# Autodesk Inventor assembly: suspensionUnitMirrored
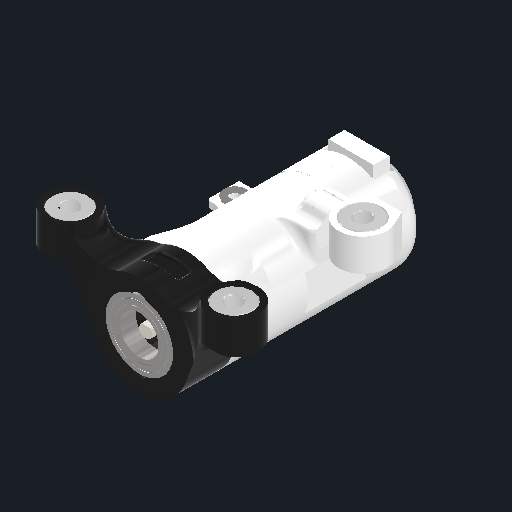
[picture p0: Inventor's stored thumbnail of the model, 512x512]
Saved by Autodesk Inventor 2025 (Build 290162000, 162)
## iProperties
Created: 2023-07-03
Part Number: suspensionUnitMirrored
Document SubType Name: Assembly
Designer: khrip
Mass: 81.1486 g
Surface Area: 305.3 cm^2
Volume: 59.2334 cm^3
Density: 1.36998 g/cm^3
Author: khrip
## Documents named in this file (13)
- H:\Potamon\OutdatedVersions\suspensionUnit\suspensionUnitMirrored.iam
- H:\Potamon\OutdatedVersions\suspensionUnit\servo.ipt
- H:\Potamon\OutdatedVersions\suspensionUnit\servoCushion.ipt
- H:\Potamon\OutdatedVersions\suspensionUnit\servoCushionSleeveMirrored.ipt
- C:\Users\khrip\OneDrive\Документы\Inventor\Content Center Files\R2023\ru-RU\GOST 17475-80 (2)\Винт 2.M3-6gx12 ГОСТ 17475-80.ipt
- H:\Potamon\OutdatedVersions\suspensionUnit\sleeve.ipt
- C:\Users\khrip\OneDrive\Документы\Inventor\Content Center Files\R2023\ru-RU\BS EN ISO 7045 H\EN ISO 7045 - M3 x 10 - 4.8 - H(1).ipt
- C:\Users\khrip\Documents\Inventor\Content Center Files\R2025\ru-RU\GOST 11371-78  A\Шайба 3 ГОСТ 11371-78.ipt
- C:\Users\khrip\OneDrive\Документы\Inventor\Content Center Files\R2023\ru-RU\DIN 934\DIN 934 - M3 x 0,5.ipt
- H:\Potamon\OutdatedVersions\suspensionUnit\bearing.ipt
- C:\Users\khrip\OneDrive\Документы\Inventor\Content Center Files\R2023\ru-RU\DIN 913\DIN 913 - M3 x 4.ipt
- H:\Potamon\OutdatedVersions\suspensionUnit\EncCoverHalf.ipt
- H:\Potamon\OutdatedVersions\suspensionUnit\EncCoverHalfMirrored.ipt
## Components (15 placed, 12 different names)
1. servo:1 — Совмещение:3, Совмещение:5, Совмещение:6, Совмещение:7, Совмещение:27, Совмещение:28, Угол:1, Совмещение:30
2. servoCushion:1 — Совмещение:1, Совмещение:2, Совмещение:4, Совмещение:5, Совмещение:6, Совмещение:7, Совмещение:8, Совмещение:9, Совмещение:12, Совмещение:13, Совмещение:14, Совмещение:15, Совмещение:22, Совмещение:23
3. servoCushionSleeveMirroredMirrored:1 — Совмещение:1, Совмещение:2, Совмещение:3, Совмещение:4, Совмещение:10, Совмещение:11, Совмещение:16, Совмещение:17, Совмещение:19, Совмещение:29, Совмещение:32
4. Винт 2 ГОСТ 17475-80 M3 x 12:1 — Совмещение:8
5. Винт 2 ГОСТ 17475-80 M3 x 12:2 — Совмещение:9
6. sleeve:1 — Совмещение:12, Совмещение:13
7. sleeve:2 — Совмещение:14, Совмещение:15
8. sleeve:3 — Совмещение:10, Совмещение:11
9. BS EN ISO 7045 H - метрическая M3 x 10 - 4.8 - H:1 — Совмещение:16, Совмещение:17, Совмещение:18, Совмещение:20
10. Шайба  ГОСТ 11371-78 3,2:1 — Совмещение:18, Совмещение:19, Совмещение:21
11. DIN 934 - заменено на DIN EN 24032/28673/28674 M3:1 — Совмещение:20, Совмещение:21
12. bearing:1 — Совмещение:22, Совмещение:23
13. DIN 913 M3 x 4:1 — Совмещение:27
14. EncCoverHalf:1 — Совмещение:28, Угол:1, Совмещение:29, Совмещение:31
15. EncCoverHalfMirrored:1 — Совмещение:30, Совмещение:31, Совмещение:32
## Relationships (30: Mate 29, Angle 1)
- Совмещение:1 [Mate]: servoCushion:1 ↔ servoCushionSleeveMirroredMirrored:1
- Совмещение:2 [Mate]: servoCushion:1 ↔ servoCushionSleeveMirroredMirrored:1
- Совмещение:3 [Mate]: servo:1 ↔ servoCushionSleeveMirroredMirrored:1
- Совмещение:4 [Mate]: servoCushion:1 ↔ servoCushionSleeveMirroredMirrored:1
- Совмещение:5 [Mate]: servo:1 ↔ servoCushion:1
- Совмещение:6 [Mate]: servo:1 ↔ servoCushion:1
- Совмещение:7 [Mate]: servo:1 ↔ servoCushion:1
- Совмещение:8 [Mate]: servoCushion:1 ↔ Винт 2 ГОСТ 17475-80 M3 x 12:1
- Совмещение:9 [Mate]: servoCushion:1 ↔ Винт 2 ГОСТ 17475-80 M3 x 12:2
- Совмещение:10 [Mate]: servoCushionSleeveMirroredMirrored:1 ↔ sleeve:3
- Совмещение:11 [Mate]: servoCushionSleeveMirroredMirrored:1 ↔ sleeve:3
- Совмещение:12 [Mate]: servoCushion:1 ↔ sleeve:1
- Совмещение:13 [Mate]: servoCushion:1 ↔ sleeve:1
- Совмещение:14 [Mate]: servoCushion:1 ↔ sleeve:2
- Совмещение:15 [Mate]: servoCushion:1 ↔ sleeve:2
- Совмещение:16 [Mate]: servoCushionSleeveMirroredMirrored:1 ↔ BS EN ISO 7045 H - метрическая M3 x 10 - 4.8 - H:1
- Совмещение:17 [Mate]: servoCushionSleeveMirroredMirrored:1 ↔ BS EN ISO 7045 H - метрическая M3 x 10 - 4.8 - H:1
- Совмещение:18 [Mate]: BS EN ISO 7045 H - метрическая M3 x 10 - 4.8 - H:1 ↔ Шайба  ГОСТ 11371-78 3,2:1
- Совмещение:19 [Mate]: servoCushionSleeveMirroredMirrored:1 ↔ Шайба  ГОСТ 11371-78 3,2:1
- Совмещение:20 [Mate]: BS EN ISO 7045 H - метрическая M3 x 10 - 4.8 - H:1 ↔ DIN 934 - заменено на DIN EN 24032/28673/28674 M3:1
- Совмещение:21 [Mate]: Шайба  ГОСТ 11371-78 3,2:1 ↔ DIN 934 - заменено на DIN EN 24032/28673/28674 M3:1
- Совмещение:22 [Mate]: servoCushion:1 ↔ bearing:1
- Совмещение:23 [Mate]: servoCushion:1 ↔ bearing:1
- Совмещение:27 [Mate]: servo:1 ↔ DIN 913 M3 x 4:1
- Совмещение:28 [Mate]: servo:1 ↔ EncCoverHalf:1
- Угол:1 [Angle] (180 deg): servo:1 ↔ EncCoverHalf:1
- Совмещение:29 [Mate]: servoCushionSleeveMirroredMirrored:1 ↔ EncCoverHalf:1
- Совмещение:30 [Mate]: servo:1 ↔ EncCoverHalfMirrored:1
- Совмещение:31 [Mate]: EncCoverHalf:1 ↔ EncCoverHalfMirrored:1
- Совмещение:32 [Mate]: servoCushionSleeveMirroredMirrored:1 ↔ EncCoverHalfMirrored:1
